# Autodesk Inventor assembly: bett_sitzbank
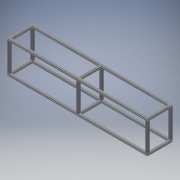
[picture p0: Inventor's stored thumbnail of the model, 180x180]
Saved by Autodesk Inventor 2018 (Build 220112000, 112)
## iProperties
Created: 2020-03-29
Part Number: bett_sitzbank
Material: Generisch
Document SubType Name: Assembly
Designer: wepet
Author: wepet
## Documents named in this file (4)
- C:\Users\wepet\Downloads\anhaenger\bett_sitzbank.iam
- C:\Users\wepet\Downloads\anhaenger\item_30x30_30cm.ipt
- C:\Users\wepet\Downloads\anhaenger\item_30x30_40cm.ipt
- C:\Users\wepet\Downloads\anhaenger\item_30x30_200cm.ipt
## Components (16 placed, 3 different names)
1. item_30x30_30cm:1 — Fluchtend:2, Passend:3, Fluchtend:3, Passend:5
2. item_30x30_40cm:1 — Fluchtend:4, Passend:4, Fluchtend:5, Passend:6, Fluchtend:15
3. item_30x30_200cm:1 — Passend:1, Passend:2, Fluchtend:1, Fluchtend:2, Passend:3, Fluchtend:3, Fluchtend:4, Passend:4, Fluchtend:5, Fluchtend:6, Fluchtend:7, Fluchtend:8, Fluchtend:9, Fluchtend:10
4. item_30x30_200cm:2 — Fluchtend:6, Fluchtend:7, Passend:5, Fluchtend:12, Fluchtend:13, Fluchtend:14, Passend:7
5. item_30x30_200cm:3 — Fluchtend:8, Fluchtend:9, Passend:6, Fluchtend:11, Fluchtend:16, Passend:8, Fluchtend:23, Fluchtend:25, Fluchtend:32, Fluchtend:33
6. item_30x30_200cm:4 — Fluchtend:10, Fluchtend:11, Fluchtend:12, Fluchtend:24
7. item_30x30_40cm:2 — Fluchtend:13, Fluchtend:14, Passend:7
8. item_30x30_30cm:2 — Fluchtend:15, Fluchtend:16, Passend:8, Fluchtend:34
9. item_30x30_30cm:3 — Fluchtend:20, Fluchtend:22, Passend:11, Passend:12
10. item_30x30_40cm:3 — Fluchtend:19, Fluchtend:21, Passend:12, Fluchtend:25
11. item_30x30_40cm:4 — Fluchtend:18, Fluchtend:21, Passend:9, Passend:10, Passend:11
12. item_30x30_30cm:4 — Fluchtend:18, Fluchtend:19, Fluchtend:20, Fluchtend:22, Passend:9, Passend:10, Fluchtend:23, Fluchtend:24
13. item_30x30_30cm:5
14. item_30x30_40cm:5 — Fluchtend:32
15. item_30x30_40cm:6
16. item_30x30_30cm:6 — Fluchtend:33, Fluchtend:34
## Relationships (50: Flush 34, Mate 16)
- Passend:1 [Mate]: item_30x30_200cm:1
- Passend:2 [Mate]: item_30x30_200cm:1
- Fluchtend:1 [Flush]: item_30x30_200cm:1
- Fluchtend:2 [Flush]: item_30x30_30cm:1 ↔ item_30x30_200cm:1
- Passend:3 [Mate]: item_30x30_30cm:1 ↔ item_30x30_200cm:1
- Fluchtend:3 [Flush]: item_30x30_30cm:1 ↔ item_30x30_200cm:1
- Fluchtend:4 [Flush]: item_30x30_40cm:1 ↔ item_30x30_200cm:1
- Passend:4 [Mate]: item_30x30_40cm:1 ↔ item_30x30_200cm:1
- Fluchtend:5 [Flush]: item_30x30_40cm:1 ↔ item_30x30_200cm:1
- Fluchtend:6 [Flush]: item_30x30_200cm:1 ↔ item_30x30_200cm:2
- Fluchtend:7 [Flush]: item_30x30_200cm:1 ↔ item_30x30_200cm:2
- Passend:5 [Mate]: item_30x30_30cm:1 ↔ item_30x30_200cm:2
- Fluchtend:8 [Flush]: item_30x30_200cm:1 ↔ item_30x30_200cm:3
- Fluchtend:9 [Flush]: item_30x30_200cm:1 ↔ item_30x30_200cm:3
- Passend:6 [Mate]: item_30x30_40cm:1 ↔ item_30x30_200cm:3
- Fluchtend:10 [Flush]: item_30x30_200cm:1 ↔ item_30x30_200cm:4
- Fluchtend:11 [Flush]: item_30x30_200cm:3 ↔ item_30x30_200cm:4
- Fluchtend:12 [Flush]: item_30x30_200cm:2 ↔ item_30x30_200cm:4
- Fluchtend:13 [Flush]: item_30x30_200cm:2 ↔ item_30x30_40cm:2
- Fluchtend:14 [Flush]: item_30x30_200cm:2 ↔ item_30x30_40cm:2
- Passend:7 [Mate]: item_30x30_200cm:2 ↔ item_30x30_40cm:2
- Fluchtend:15 [Flush]: item_30x30_40cm:1 ↔ item_30x30_30cm:2
- Fluchtend:16 [Flush]: item_30x30_200cm:3 ↔ item_30x30_30cm:2
- Passend:8 [Mate]: item_30x30_200cm:3 ↔ item_30x30_30cm:2
- [Flush]: item_30x30_40cm:3 ↔ item_30x30_30cm:4
- Fluchtend:18 [Flush]: item_30x30_40cm:4 ↔ item_30x30_30cm:4
- Fluchtend:19 [Flush]: item_30x30_40cm:3 ↔ item_30x30_30cm:4
- Fluchtend:20 [Flush]: item_30x30_30cm:3 ↔ item_30x30_30cm:4
- Fluchtend:21 [Flush]: item_30x30_40cm:3 ↔ item_30x30_40cm:4
- Fluchtend:22 [Flush]: item_30x30_30cm:3 ↔ item_30x30_30cm:4
- Passend:9 [Mate]: item_30x30_40cm:4 ↔ item_30x30_30cm:4
- Passend:10 [Mate]: item_30x30_40cm:4 ↔ item_30x30_30cm:4
- Passend:11 [Mate]: item_30x30_30cm:3 ↔ item_30x30_40cm:4
- Passend:12 [Mate]: item_30x30_30cm:3 ↔ item_30x30_40cm:3
- Fluchtend:23 [Flush]: item_30x30_200cm:3 ↔ item_30x30_30cm:4
- Fluchtend:24 [Flush]: item_30x30_200cm:4 ↔ item_30x30_30cm:4
- Fluchtend:25 [Flush]: item_30x30_200cm:3 ↔ item_30x30_40cm:3
- [Flush]: item_30x30_40cm:5 ↔ item_30x30_30cm:6
- [Flush]: item_30x30_40cm:6 ↔ item_30x30_30cm:6
- [Flush]: item_30x30_40cm:5 ↔ item_30x30_30cm:6
- [Flush]: item_30x30_30cm:5 ↔ item_30x30_30cm:6
- [Flush]: item_30x30_40cm:5 ↔ item_30x30_40cm:6
- [Flush]: item_30x30_30cm:5 ↔ item_30x30_30cm:6
- [Mate]: item_30x30_40cm:6 ↔ item_30x30_30cm:6
- [Mate]: item_30x30_40cm:6 ↔ item_30x30_30cm:6
- [Mate]: item_30x30_30cm:5 ↔ item_30x30_40cm:6
- [Mate]: item_30x30_30cm:5 ↔ item_30x30_40cm:5
- Fluchtend:32 [Flush]: item_30x30_200cm:3 ↔ item_30x30_40cm:5
- Fluchtend:33 [Flush]: item_30x30_200cm:3 ↔ item_30x30_30cm:6
- Fluchtend:34 [Flush] (98.5 mm): item_30x30_30cm:2 ↔ item_30x30_30cm:6
## Named parameters: d24_d21 = 0 mm, d37_d26 = 0 mm, d38_d27 = 0 mm, d39_d28 = 0 mm, d40_d29 = 0 mm, d41_d30 = 0 mm, d42_d31 = 0 mm, d43_d32 = 0 mm, d44_d33 = 0 mm, d45_d24_d21 = 0 mm, d46_d25 = 0 mm
